# Autodesk Inventor assembly: 組合檔
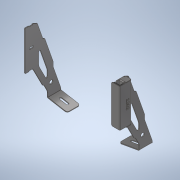
[picture p0: Inventor's stored thumbnail of the model, 180x180]
Saved by Autodesk Inventor 2020 (Build 240168000, 168)
## iProperties
Created: 2015-11-28
Part Number: 組合檔
Document SubType Name: Assembly
Designer: 設計製圖
Author: 設計製圖
## Documents named in this file (18)
- D:\資料庫\設計-3D Project\【May club 】\得利卡-車頂燈架\模型、圖面\短-車頂燈架-組合(#11.02).iam
- D:\資料庫\設計-3D Project\【 鐵蹄 】\------鐵蹄工廠素材------ -\拉帽-M8.ipt
- D:\資料庫\設計-3D Project\【May club 】\得利卡-車頂燈架\模型、圖面\焊接組件-1(#11.02).ipt
- D:\資料庫\設計-3D Project\材料庫\【螺絲】\止付螺絲\止付螺絲-M8-20.ipt
- D:\資料庫\設計-3D Project\【May club 】\得利卡-車頂燈架\模型、圖面\車身圖.ipt
- D:\資料庫\設計-3D Project\【May club 】\得利卡-車頂燈架\模型、圖面\吊架組件-ㄇ槽(#11.02).ipt
- D:\資料庫\設計-3D Project\【May club 】\得利卡-車頂燈架\模型、圖面\吊架-短(R)(#11.02).ipt
- D:\資料庫\設計-3D Project\【May club 】\得利卡-車頂燈架\模型、圖面\焊接組件-2(#11.02).ipt
- D:\資料庫\設計-3D Project\【May club 】\得利卡-車頂燈架\模型、圖面\得利卡-車頂導水槽.ipt
- D:\資料庫\設計-3D Project\材料庫\螺帽\白鐵-六角螺帽-M6.ipt
- D:\資料庫\設計-3D Project\【May club 】\得利卡-車頂燈架\模型、圖面\吊架-短(L)(#11.02)_MIR.ipt
- D:\資料庫\設計-3D Project\材料庫\【螺絲】\外六角螺絲\白鐵-外六角  M6-20.ipt
- D:\資料庫\設計-3D Project\材料庫\【華司】\白鐵-平面華司-7-16-2t.ipt
- D:\資料庫\設計-3D Project\材料庫\【華司】\彈簧華司\白鐵-彈簧華司-6.ipt
- D:\資料庫\設計-3D Project\【May club 】\得利卡-車頂燈架\模型、圖面\短-車頂燈架-組合(#11.02)-生產圖面_21.11.26\製程筆記\封邊條 ( 平光黑 ) - 130L.ipt
- D:\資料庫\設計-3D Project\【May club 】\得利卡-車頂燈架\模型、圖面\短-車頂燈架-組合(#11.02)-生產圖面_21.11.26\製程筆記\背膠海綿eva 6T -  15W x 125L.ipt
- D:\資料庫\設計-3D Project\【May club 】\得利卡-車頂燈架\模型、圖面\短-車頂燈架-組合(#11.02)-生產圖面_21.11.26\製程筆記\背膠海綿eva 3T -  25W x 125L.ipt
- D:\資料庫\設計-3D Project\【May club 】\得利卡-車頂燈架\模型、圖面\短-車頂燈架-組合(#11.02)-生產圖面_21.11.26\製程筆記\背膠海綿eva 3T -  10W x 125L.ipt
## Components (19 placed, 17 different names)
1. 拉帽-M8:2 — 齊平:6, 貼合:15, 貼合:32, 貼合:38
2. 拉帽-M8:1 — 齊平:6, 貼合:15, 貼合:17, 貼合:31, 貼合:37
3. 白鐵-六角螺帽-M6:1 — 貼合:44, 貼合:45, 齊平:15, 貼合:46
4. 吊架組件-ㄇ槽(#11.02):1 — 貼合:17, 貼合:37, 貼合:38, 貼合:40, 齊平:14, 貼合:41, 貼合:18, 齊平:13, 齊平:16, 貼合:57, 貼合:58, 貼合:59, 貼合:60, 貼合:61
5. 吊架-短(R)(#11.02):1 — 貼合:3, 貼合:4, 齊平:1, 貼合:18, 貼合:23, 貼合:26, 貼合:33, 齊平:17, 貼合:50, 齊平:18, 貼合:56
6. 焊接組件-1(#11.02):1 — 貼合:23, 貼合:26, 齊平:13, 齊平:16, 貼合:53, 齊平:18, 貼合:54, 貼合:55
7. 焊接組件-2(#11.02):1 — 貼合:40, 齊平:14, 貼合:41, 貼合:44, 貼合:45, 齊平:15
8. 吊架-短(L)(#11.02)_MIR:1 — 貼合:47
9. 得利卡-車頂導水槽:1
10. 車身圖:1 — 貼合:33
11. 背膠海綿eva 6T -  15W x 125L:1 — 貼合:54, 貼合:55, 貼合:56
12. 背膠海綿eva 3T -  25W x 125L:1 — 貼合:57, 貼合:58, 貼合:59, 貼合:62
13. 背膠海綿eva 3T -  10W x 125L:1 — 貼合:60, 貼合:61, 貼合:62
14. 白鐵-彈簧華司-6:1 — 貼合:49, 貼合:51, 貼合:52
15. 白鐵-平面華司-7-16-2t:1 — 貼合:48, 貼合:50, 貼合:51
16. 白鐵-外六角  M6-20:1 — 貼合:46, 貼合:48, 貼合:49, 貼合:52
17. 封邊條 ( 平光黑 ) - 130L:1 — 貼合:3, 貼合:4, 齊平:1
18. 止付螺絲-M8-20:1 — 齊平:12, 貼合:31, 貼合:53
19. 止付螺絲-M8-20:2 — 齊平:12, 貼合:32
## Relationships (42: Mate 33, Flush 9)
- 貼合:3 [Mate]: 吊架-短(R)(#11.02):1 ↔ 封邊條 ( 平光黑 ) - 130L:1
- 貼合:4 [Mate]: 吊架-短(R)(#11.02):1 ↔ 封邊條 ( 平光黑 ) - 130L:1
- 齊平:1 [Flush]: 吊架-短(R)(#11.02):1 ↔ 封邊條 ( 平光黑 ) - 130L:1
- 齊平:6 [Flush]: 拉帽-M8:2 ↔ 拉帽-M8:1
- 貼合:15 [Mate]: 拉帽-M8:2 ↔ 拉帽-M8:1
- 貼合:17 [Mate]: 拉帽-M8:1 ↔ 吊架組件-ㄇ槽(#11.02):1
- 貼合:23 [Mate]: 吊架-短(R)(#11.02):1 ↔ 焊接組件-1(#11.02):1
- 貼合:26 [Mate]: 吊架-短(R)(#11.02):1 ↔ 焊接組件-1(#11.02):1
- 齊平:12 [Flush]: 止付螺絲-M8-20:1 ↔ 止付螺絲-M8-20:2
- 貼合:31 [Mate]: 拉帽-M8:1 ↔ 止付螺絲-M8-20:1
- 貼合:32 [Mate]: 拉帽-M8:2 ↔ 止付螺絲-M8-20:2
- 貼合:33 [Mate]: 吊架-短(R)(#11.02):1 ↔ 車身圖:1
- 貼合:37 [Mate]: 拉帽-M8:1 ↔ 吊架組件-ㄇ槽(#11.02):1
- 貼合:38 [Mate]: 拉帽-M8:2 ↔ 吊架組件-ㄇ槽(#11.02):1
- 貼合:40 [Mate]: 吊架組件-ㄇ槽(#11.02):1 ↔ 焊接組件-2(#11.02):1
- 齊平:14 [Flush]: 吊架組件-ㄇ槽(#11.02):1 ↔ 焊接組件-2(#11.02):1
- 貼合:41 [Mate]: 吊架組件-ㄇ槽(#11.02):1 ↔ 焊接組件-2(#11.02):1
- 貼合:18 [Mate]: 吊架組件-ㄇ槽(#11.02):1 ↔ 吊架-短(R)(#11.02):1
- 齊平:13 [Flush]: 吊架組件-ㄇ槽(#11.02):1 ↔ 焊接組件-1(#11.02):1
- 貼合:44 [Mate]: 白鐵-六角螺帽-M6:1 ↔ 焊接組件-2(#11.02):1
- 貼合:45 [Mate]: 白鐵-六角螺帽-M6:1 ↔ 焊接組件-2(#11.02):1
- 齊平:15 [Flush]: 白鐵-六角螺帽-M6:1 ↔ 焊接組件-2(#11.02):1
- 貼合:46 [Mate]: 白鐵-六角螺帽-M6:1 ↔ 白鐵-外六角  M6-20:1
- 齊平:16 [Flush]: 吊架組件-ㄇ槽(#11.02):1 ↔ 焊接組件-1(#11.02):1
- 齊平:17 [Flush] (150 mm): 吊架-短(R)(#11.02):1
- 貼合:47 [Mate] (150 mm): 吊架-短(L)(#11.02)_MIR:1
- 貼合:48 [Mate]: 白鐵-平面華司-7-16-2t:1 ↔ 白鐵-外六角  M6-20:1
- 貼合:49 [Mate]: 白鐵-彈簧華司-6:1 ↔ 白鐵-外六角  M6-20:1
- 貼合:50 [Mate]: 吊架-短(R)(#11.02):1 ↔ 白鐵-平面華司-7-16-2t:1
- 貼合:51 [Mate]: 白鐵-彈簧華司-6:1 ↔ 白鐵-平面華司-7-16-2t:1
- 貼合:52 [Mate]: 白鐵-彈簧華司-6:1 ↔ 白鐵-外六角  M6-20:1
- 貼合:53 [Mate]: 焊接組件-1(#11.02):1 ↔ 止付螺絲-M8-20:1
- 齊平:18 [Flush]: 吊架-短(R)(#11.02):1 ↔ 焊接組件-1(#11.02):1
- 貼合:54 [Mate]: 焊接組件-1(#11.02):1 ↔ 背膠海綿eva 6T -  15W x 125L:1
- 貼合:55 [Mate]: 焊接組件-1(#11.02):1 ↔ 背膠海綿eva 6T -  15W x 125L:1
- 貼合:56 [Mate]: 吊架-短(R)(#11.02):1 ↔ 背膠海綿eva 6T -  15W x 125L:1
- 貼合:57 [Mate]: 吊架組件-ㄇ槽(#11.02):1 ↔ 背膠海綿eva 3T -  25W x 125L:1
- 貼合:58 [Mate]: 吊架組件-ㄇ槽(#11.02):1 ↔ 背膠海綿eva 3T -  25W x 125L:1
- 貼合:59 [Mate]: 吊架組件-ㄇ槽(#11.02):1 ↔ 背膠海綿eva 3T -  25W x 125L:1
- 貼合:60 [Mate]: 吊架組件-ㄇ槽(#11.02):1 ↔ 背膠海綿eva 3T -  10W x 125L:1
- 貼合:61 [Mate]: 吊架組件-ㄇ槽(#11.02):1 ↔ 背膠海綿eva 3T -  10W x 125L:1
- 貼合:62 [Mate]: 背膠海綿eva 3T -  25W x 125L:1 ↔ 背膠海綿eva 3T -  10W x 125L:1
